# Autodesk Inventor assembly: KabineChassis
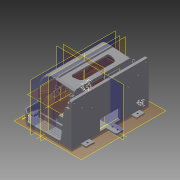
[picture p0: Inventor's stored thumbnail of the model, 180x180]
Saved by Autodesk Inventor 2015 (Build 190159000, 159)
## iProperties
Created: 2018-10-29
Part Number: KabineChassis
Document SubType Name: Assembly
Designer: Boris
Author: Boris
## Documents named in this file (4)
- D:\Wisag Hiserv\HiSERV Smart Drive\WorkOrder\3D - Teile\STL\KabineChassis.iam
- D:\Wisag Hiserv\HiSERV Smart Drive\WorkOrder\3D - Teile\KabineChassis.ipt
- D:\Wisag Hiserv\HiSERV Smart Drive\WorkOrder\3D - Teile\Lenkrad.ipt
- D:\Wisag Hiserv\HiSERV Smart Drive\WorkOrder\3D - Teile\KabineTeil1.ipt
## Components (3 placed, 3 different names)
1. KabineChassis:1 — Einfügen:2, Einfügen:3, Einfügen:4
2. Lenkrad:1 — Einfügen:2
3. KabineTeil1:1 — Einfügen:3, Einfügen:4
## Relationships (3: Insert 3)
- Einfügen:2 [Insert] (-2.5 mm): KabineChassis:1 ↔ Lenkrad:1
- Einfügen:3 [Insert] (-5 mm): KabineChassis:1 ↔ KabineTeil1:1
- Einfügen:4 [Insert] (-5 mm): KabineChassis:1 ↔ KabineTeil1:1
